# Autodesk Inventor assembly: 200-50-BOGIE-ASM-01
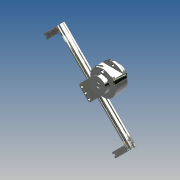
[picture p0: Inventor's stored thumbnail of the model, 180x180]
Saved by Autodesk Inventor 2018.2 (Build 222227000, 227)
## iProperties
Manager: feesmrt
Company: FRANC0R
Created: 2017-12-10
Part Number: 200-50-BOGIE-ASM-01
Material: Generisch
Document SubType Name: Assembly
Designer: feesmrt
Project: Rescue Robot
Cost Center: -
Description: Bogie Assembly
Engineer: feesmrt
Authority: feesmrt
Stock Number: 200-50-BOGIE-ASM-01
Author: feesmrt
Title: Bogie Assembly
Subject: Rescue Robot
Revision Number: 1
## Documents named in this file (3)
- D:\Programmierung\FRANC0R\CAD\02-Rocker-Bogie-Robot\200-ROCKER-BOGIE\200-50-BOGIE-ASM-01.iam
- D:\Programmierung\FRANC0R\CAD\02-Rocker-Bogie-Robot\200-ROCKER-BOGIE\200-30-BOGIE-BEARING-ASM-01.iam
- D:\Programmierung\FRANC0R\CAD\02-Rocker-Bogie-Robot\200-ROCKER-BOGIE\200-40-BOGIE-CONNECTOR-ASM-01.iam
## Components (2 placed, 2 different names)
1. 200-30-BOGIE-BEARING-ASM-01:1 [sub-assembly] — Winkel:1, Passend:2, Passend:3
2. 200-40-BOGIE-CONNECTOR-ASM-01:1 [sub-assembly] — Winkel:1, Passend:2, Passend:3
## Relationships (3: Mate 2, Angle 1)
- Winkel:1 [Angle] (45 deg): 200-30-BOGIE-BEARING-ASM-01:1 ↔ 200-40-BOGIE-CONNECTOR-ASM-01:1
- Passend:2 [Mate]: 200-30-BOGIE-BEARING-ASM-01:1 ↔ 200-40-BOGIE-CONNECTOR-ASM-01:1
- Passend:3 [Mate]: 200-30-BOGIE-BEARING-ASM-01:1 ↔ 200-40-BOGIE-CONNECTOR-ASM-01:1
